# Autodesk Inventor assembly: ModuloLavaplatos_2
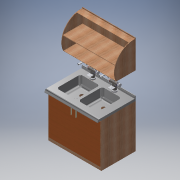
[picture p0: Inventor's stored thumbnail of the model, 180x180]
Saved by Autodesk Inventor 2016 (Build 200138000, 138)
## iProperties
Created: 2015-11-25
Part Number: ModuloLavaplatos_2
Document SubType Name: Assembly
Designer: Daniela
Author: Daniela
## Documents named in this file (6)
- D:\Documents\Carrera\11.Semeste_II_2015\Computacion_grafica\Proyecto\COCINA_FINAL\Cocina\ModuloLavaplatos_2.iam
- D:\Documents\Carrera\11.Semeste_II_2015\Computacion_grafica\Proyecto\COCINA_FINAL\Cocina\base_lavaplatos.ipt
- D:\Documents\Carrera\11.Semeste_II_2015\Computacion_grafica\Proyecto\COCINA_FINAL\Cocina\grifo.ipt
- D:\Documents\Carrera\11.Semeste_II_2015\Computacion_grafica\Proyecto\COCINA_FINAL\Cocina\puerta_lavaplatos.ipt
- D:\Documents\Carrera\11.Semeste_II_2015\Computacion_grafica\Proyecto\COCINA_FINAL\Cocina\manija.ipt
- D:\Documents\Carrera\11.Semeste_II_2015\Computacion_grafica\Proyecto\COCINA_FINAL\Cocina\lavaplatos_2.ipt
## Components (8 placed, 5 different names)
1. base_lavaplatos:1 — Mate:5, Mate:6, Mate:7, Mate:14, Flush:5, Flush:6
2. grifo:1 — Mate:16, Mate:17
3. puerta_lavaplatos:1 — Flush:3, Flush:4, Mate:4, Mate:9, Mate:11, Mate:12
4. puerta_lavaplatos:2 — Flush:3, Flush:4, Mate:4, Mate:5, Mate:6, Mate:7, Mate:8, Mate:10, Mate:13
5. manija:1 — Mate:8, Mate:10, Mate:13
6. manija:2 — Mate:9, Mate:11, Mate:12
7. lavaplatos_2:1 — Mate:14, Flush:5, Flush:6, Mate:15, Mate:16, Mate:17, Mate:18
8. grifo:2 — Mate:15, Mate:18
## Relationships (19: Mate 15, Flush 4)
- Flush:3: puerta_lavaplatos:1 ↔ puerta_lavaplatos:2
- Flush:4: puerta_lavaplatos:1 ↔ puerta_lavaplatos:2
- Mate:4: puerta_lavaplatos:1 ↔ puerta_lavaplatos:2
- Mate:5: base_lavaplatos:1 ↔ puerta_lavaplatos:2
- Mate:6 (-10 mm): base_lavaplatos:1 ↔ puerta_lavaplatos:2
- Mate:7 (-10 mm): base_lavaplatos:1 ↔ puerta_lavaplatos:2
- Mate:8: puerta_lavaplatos:2 ↔ manija:1
- Mate:9: puerta_lavaplatos:1 ↔ manija:2
- Mate:10: puerta_lavaplatos:2 ↔ manija:1
- Mate:11: puerta_lavaplatos:1 ↔ manija:2
- Mate:12: puerta_lavaplatos:1 ↔ manija:2
- Mate:13: puerta_lavaplatos:2 ↔ manija:1
- Mate:14: base_lavaplatos:1 ↔ lavaplatos_2:1
- Flush:5: base_lavaplatos:1 ↔ lavaplatos_2:1
- Flush:6: base_lavaplatos:1 ↔ lavaplatos_2:1
- Mate:15: lavaplatos_2:1 ↔ grifo:2
- Mate:16: grifo:1 ↔ lavaplatos_2:1
- Mate:17: grifo:1 ↔ lavaplatos_2:1
- Mate:18: lavaplatos_2:1 ↔ grifo:2
